# Autodesk Inventor assembly: Frame
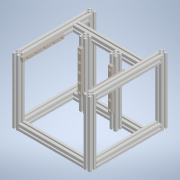
[picture p0: Inventor's stored thumbnail of the model, 180x180]
Saved by Autodesk Inventor 2022 (Build 260153000, 153)
## iProperties
Created: 2021-11-24
Part Number: Frame
Document SubType Name: Assembly
Designer: yuto6
Author: yuto6
## Documents named in this file (3)
- C:\Users\yuto6\Documents\My3DPrinter\CAD\Asm\Frame.iam
- C:\Users\yuto6\Documents\My3DPrinter\CAD\Parts\HFS3-1515-150.ipt
- C:\Users\yuto6\Documents\My3DPrinter\CAD\Parts\Linear Guide Rail LML9B.ipt
## Components (17 placed, 2 different names)
1. HFS3-1515-150:1 — メイト:1, メイト:3, フラッシュ:5, フラッシュ:6, フラッシュ:7, フラッシュ:8, フラッシュ:14, フラッシュ:15
2. HFS3-1515-150:2 — メイト:2, メイト:8, フラッシュ:1, フラッシュ:2, フラッシュ:3, フラッシュ:4, フラッシュ:12, フラッシュ:13
3. HFS3-1515-150:3 — メイト:7, メイト:10
4. HFS3-1515-150:4 — メイト:4, フラッシュ:9, フラッシュ:10, メイト:11
5. HFS3-1515-150:5 — メイト:1, メイト:2, フラッシュ:3, フラッシュ:4, フラッシュ:5, フラッシュ:8
6. HFS3-1515-150:7 — メイト:7, メイト:8, フラッシュ:1, フラッシュ:2, メイト:9, フラッシュ:11
7. HFS3-1515-150:8 — メイト:3, メイト:4, フラッシュ:6, フラッシュ:7, フラッシュ:9, フラッシュ:10
8. HFS3-1515-150:9 — メイト:9, フラッシュ:11, フラッシュ:17
9. HFS3-1515-150:10 — フラッシュ:14, フラッシュ:15, メイト:11, フラッシュ:16, メイト:13, フラッシュ:18
10. HFS3-1515-150:11 — フラッシュ:12, フラッシュ:13, メイト:10, メイト:12, メイト:14, フラッシュ:19
11. HFS3-1515-150:12 — フラッシュ:16, メイト:12, フラッシュ:17, メイト:15, メイト:16, フラッシュ:21, フラッシュ:22
12. Linear Guide Rail LML9B:1 — メイト:13, フラッシュ:18, フラッシュ:20
13. Linear Guide Rail LML9B:2 — メイト:14, フラッシュ:19, フラッシュ:20
14. HFS3-1515-150:13 — メイト:15, フラッシュ:21, メイト:17, フラッシュ:24
15. HFS3-1515-150:14 — メイト:16, フラッシュ:22, メイト:18, フラッシュ:23
16. Linear Guide Rail LML9B:3 — メイト:17, フラッシュ:24, フラッシュ:25
17. Linear Guide Rail LML9B:4 — メイト:18, フラッシュ:23, フラッシュ:25
## Relationships (41: Flush 25, Mate 16)
- メイト:1 [Mate]: HFS3-1515-150:1 ↔ HFS3-1515-150:5
- メイト:2 [Mate]: HFS3-1515-150:2 ↔ HFS3-1515-150:5
- メイト:3 [Mate]: HFS3-1515-150:1 ↔ HFS3-1515-150:8
- メイト:4 [Mate]: HFS3-1515-150:4 ↔ HFS3-1515-150:8
- メイト:7 [Mate]: HFS3-1515-150:3 ↔ HFS3-1515-150:7
- メイト:8 [Mate]: HFS3-1515-150:2 ↔ HFS3-1515-150:7
- フラッシュ:1 [Flush]: HFS3-1515-150:2 ↔ HFS3-1515-150:7
- フラッシュ:2 [Flush]: HFS3-1515-150:2 ↔ HFS3-1515-150:7
- フラッシュ:3 [Flush]: HFS3-1515-150:2 ↔ HFS3-1515-150:5
- フラッシュ:4 [Flush]: HFS3-1515-150:2 ↔ HFS3-1515-150:5
- フラッシュ:5 [Flush]: HFS3-1515-150:1 ↔ HFS3-1515-150:5
- フラッシュ:6 [Flush]: HFS3-1515-150:1 ↔ HFS3-1515-150:8
- フラッシュ:7 [Flush]: HFS3-1515-150:1 ↔ HFS3-1515-150:8
- フラッシュ:8 [Flush]: HFS3-1515-150:1 ↔ HFS3-1515-150:5
- フラッシュ:9 [Flush]: HFS3-1515-150:4 ↔ HFS3-1515-150:8
- フラッシュ:10 [Flush]: HFS3-1515-150:4 ↔ HFS3-1515-150:8
- メイト:9 [Mate]: HFS3-1515-150:7 ↔ HFS3-1515-150:9
- フラッシュ:11 [Flush]: HFS3-1515-150:7 ↔ HFS3-1515-150:9
- フラッシュ:12 [Flush]: HFS3-1515-150:2 ↔ HFS3-1515-150:11
- フラッシュ:13 [Flush]: HFS3-1515-150:2 ↔ HFS3-1515-150:11
- メイト:10 [Mate]: HFS3-1515-150:3 ↔ HFS3-1515-150:11
- フラッシュ:14 [Flush]: HFS3-1515-150:1 ↔ HFS3-1515-150:10
- フラッシュ:15 [Flush]: HFS3-1515-150:1 ↔ HFS3-1515-150:10
- メイト:11 [Mate]: HFS3-1515-150:4 ↔ HFS3-1515-150:10
- フラッシュ:16 [Flush]: HFS3-1515-150:10 ↔ HFS3-1515-150:12
- メイト:12 [Mate]: HFS3-1515-150:11 ↔ HFS3-1515-150:12
- フラッシュ:17 [Flush]: HFS3-1515-150:9 ↔ HFS3-1515-150:12
- メイト:13 [Mate]: HFS3-1515-150:10 ↔ Linear Guide Rail LML9B:1
- メイト:14 [Mate]: HFS3-1515-150:11 ↔ Linear Guide Rail LML9B:2
- フラッシュ:18 [Flush] (3 mm): HFS3-1515-150:10 ↔ Linear Guide Rail LML9B:1
- フラッシュ:19 [Flush] (3 mm): HFS3-1515-150:11 ↔ Linear Guide Rail LML9B:2
- フラッシュ:20 [Flush]: Linear Guide Rail LML9B:1 ↔ Linear Guide Rail LML9B:2
- メイト:15 [Mate]: HFS3-1515-150:12 ↔ HFS3-1515-150:13
- メイト:16 [Mate]: HFS3-1515-150:12 ↔ HFS3-1515-150:14
- フラッシュ:21 [Flush]: HFS3-1515-150:12 ↔ HFS3-1515-150:13
- フラッシュ:22 [Flush]: HFS3-1515-150:12 ↔ HFS3-1515-150:14
- メイト:17 [Mate]: HFS3-1515-150:13 ↔ Linear Guide Rail LML9B:3
- メイト:18 [Mate]: HFS3-1515-150:14 ↔ Linear Guide Rail LML9B:4
- フラッシュ:23 [Flush] (3 mm): HFS3-1515-150:14 ↔ Linear Guide Rail LML9B:4
- フラッシュ:24 [Flush] (3 mm): HFS3-1515-150:13 ↔ Linear Guide Rail LML9B:3
- フラッシュ:25 [Flush]: Linear Guide Rail LML9B:3 ↔ Linear Guide Rail LML9B:4
